# Autodesk Inventor assembly: pruzina
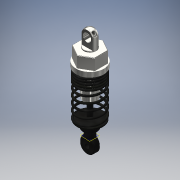
[picture p0: Inventor's stored thumbnail of the model, 180x180]
Saved by Autodesk Inventor 2016 (Build 200138000, 138)
## iProperties
Created: 2016-11-29
Part Number: pruzina
Document SubType Name: Assembly
Designer: Juraj
Author: Juraj
## Documents named in this file (4)
- C:\Users\Juraj\Documents\GitHub\Robot6x6\Terrenny robot CAD\pruzina\pruzina.iam
- C:\Users\Juraj\Documents\GitHub\Robot6x6\Terrenny robot CAD\pruzina\cast1.ipt
- C:\Users\Juraj\Documents\GitHub\Robot6x6\Terrenny robot CAD\pruzina\pruzina.ipt
- C:\Users\Juraj\Documents\GitHub\Robot6x6\Terrenny robot CAD\pruzina\cast2.ipt
## Components (3 placed, 3 different names)
1. cast1:1 — Insert:4, Mate:1
2. cast2:1 — Insert:4, Mate:2, Mate:3
3. pruzina:1 — Mate:1, Mate:2, Mate:3
## Relationships (4: Mate 3, Insert 1)
- Insert:4 (-4.1 mm): cast1:1 ↔ cast2:1
- Mate:1: cast1:1 ↔ pruzina:1
- Mate:2: cast2:1 ↔ pruzina:1
- Mate:3: cast2:1 ↔ pruzina:1
